# Autodesk Inventor assembly: All Keys
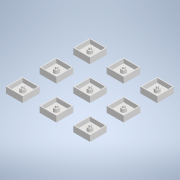
[picture p0: Inventor's stored thumbnail of the model, 180x180]
Saved by Autodesk Inventor 2021.1 (Build 251245000, 245)
## iProperties
Created: 2020-08-05
Part Number: All Keys
Document SubType Name: Assembly
Designer: adick
Author: adick
## Documents named in this file (2)
- C:\Users\adick\Documents\Kerbal Kontroller\Design\Final\3d Print\All Keys.iam
- C:\Users\adick\Documents\Kerbal Kontroller\Design\Final\Inventor\Parts\Keycaps.ipt
## Components (9 placed, 1 different names)
1. Keycaps:1
2. Keycaps:2
3. Keycaps:3
4. Keycaps:4
5. Keycaps:5
6. Keycaps:6
7. Keycaps:7
8. Keycaps:8
9. Keycaps:9
## Component patterns: (3 elements), (3 elements, first: Keycaps:1), Component Pattern 1:2 (3 elements), Component Pattern 1:3 (3 elements)
